# Autodesk Inventor assembly: SmartHome_Assembly
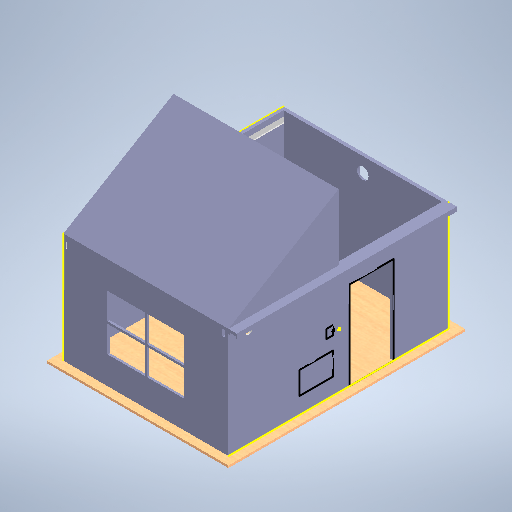
[picture p0: Inventor's stored thumbnail of the model, 512x512]
Saved by Autodesk Inventor 2026.2 (Build 302298010, 298A)
## iProperties
Created: 2026-03-19
Part Number: SmartHome_Assembly
Document SubType Name: Assembly
Designer: Patryk
Mass: 756.643 g
Surface Area: 4153.34 cm^2
Volume: 933.725 cm^3
Density: 0.810349 g/cm^3
Author: Patryk
## Documents named in this file (8)
- C:\Users\bartk\OneDrive\Dokumenty\Inventor\SmartHomeProject\SmartHome_Assembly.iam
- C:\Users\bartk\OneDrive\Dokumenty\Inventor\SmartHomeProject\MainFloorPanel.ipt
- C:\Users\bartk\OneDrive\Dokumenty\Inventor\SmartHomeProject\BackWall.ipt
- C:\Users\bartk\OneDrive\Dokumenty\Inventor\SmartHomeProject\FrontWall.ipt
- C:\Users\bartk\OneDrive\Dokumenty\Inventor\SmartHomeProject\LeftWall_Window.ipt
- C:\Users\bartk\OneDrive\Dokumenty\Inventor\SmartHomeProject\RightWall.ipt
- C:\Users\bartk\OneDrive\Dokumenty\Inventor\SmartHomeProject\PitchedRoof.ipt
- C:\Users\bartk\OneDrive\Dokumenty\Inventor\SmartHomeProject\CeilingPanel.ipt
## Components (7 placed, 7 different names)
1. MainFloorPanel:1 — Zestawiające:1, Zestawiające:2, Równoległe:3, Równoległe:4, Zestawiające:3, Równoległe:5, Zestawiające:5, Równoległe:6, Równoległe:7, Równoległe:8
2. BackWall:1 — Zestawiające:1, Zestawiające:7, Równoległe:7, Równoległe:8, Równoległe:9, Równoległe:11
3. FrontWall:1 — Zestawiające:2, Równoległe:3, Równoległe:4, Zestawiające:6, Zestawiające:8, Zestawiające:9
4. LeftWall_Window:1 — Zestawiające:3, Równoległe:5, Zestawiające:7
5. RightWall:1 — Zestawiające:5, Zestawiające:6, Równoległe:6, Równoległe:10
6. PitchedRoof:1 — Równoległe:9, Zestawiające:8, Zestawiające:10
7. CeilingPanel:1 — Zestawiające:9, Równoległe:10, Równoległe:11, Zestawiające:10
## Relationships (18: Mate 9, Flush 9)
- Zestawiające:1 [Mate]: MainFloorPanel:1 ↔ BackWall:1
- Zestawiające:2 [Mate]: MainFloorPanel:1 ↔ FrontWall:1
- Równoległe:3 [Flush] (-15 mm): MainFloorPanel:1 ↔ FrontWall:1
- Równoległe:4 [Flush] (-15 mm): MainFloorPanel:1 ↔ FrontWall:1
- Zestawiające:3 [Mate]: MainFloorPanel:1 ↔ LeftWall_Window:1
- Równoległe:5 [Flush] (-15 mm): MainFloorPanel:1 ↔ LeftWall_Window:1
- Zestawiające:5 [Mate]: MainFloorPanel:1 ↔ RightWall:1
- Zestawiające:6 [Mate]: FrontWall:1 ↔ RightWall:1
- Równoległe:6 [Flush] (-15 mm): MainFloorPanel:1 ↔ RightWall:1
- Zestawiające:7 [Mate]: BackWall:1 ↔ LeftWall_Window:1
- Równoległe:7 [Flush] (15 mm): MainFloorPanel:1 ↔ BackWall:1
- Równoległe:8 [Flush] (-15 mm): MainFloorPanel:1 ↔ BackWall:1
- Równoległe:9 [Flush]: BackWall:1 ↔ PitchedRoof:1
- Zestawiające:8 [Mate]: FrontWall:1 ↔ PitchedRoof:1
- Zestawiające:9 [Mate]: FrontWall:1 ↔ CeilingPanel:1
- Równoległe:10 [Flush]: RightWall:1 ↔ CeilingPanel:1
- Równoległe:11 [Flush]: BackWall:1 ↔ CeilingPanel:1
- Zestawiające:10 [Mate]: PitchedRoof:1 ↔ CeilingPanel:1
